# Autodesk Inventor assembly: 1Ufullsystem
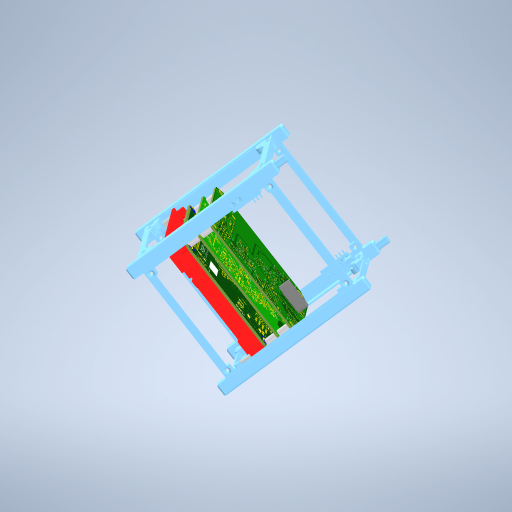
[picture p0: Inventor's stored thumbnail of the model, 512x512]
Saved by Autodesk Inventor 2024 (Build 280153000, 153)
## iProperties
Created: 2023-04-12
Part Number: 1Ufullsystem
Document SubType Name: Assembly
Designer: User
Author: User
## Documents named in this file (8)
- C:\Users\User\Documents\1UFrame\1Ufullsystem.iam
- C:\Users\User\Documents\1UFrame\ISISpace\ISIS CubeSat STS PC104 Skeleton.iam
- C:\Users\User\Documents\1UFrame\CAD_backup_frequent_files_20200629 (1)\PCB_LT_ICR.iam
- C:\Users\User\Documents\1UFrame\CAD_backup_frequent_files_20200629 (1)\PCB_LT_RX-TX.iam
- C:\Users\User\Documents\1UFrame\CAD_backup_frequent_files_20200629 (1)\PCB_LIHU.iam
- C:\Users\User\Documents\1UFrame\CAD_backup_frequent_files_20200629 (1)\standoff815mm.ipt
- C:\Users\User\Documents\1UFrame\Standoff0.335in.ipt
- C:\Users\User\Documents\1UFrame\PC104_EM-113 Assembly.iam
## Components (17 placed, 7 different names)
1. ISIS CubeSat STS PC104 Skeleton:1 [sub-assembly] — Mate:1, Mate:2, Mate:3, Mate:4
2. PCB_LT_ICR:1 [sub-assembly] — Mate:16, Mate:17, Mate:18, Mate:19, Mate:20, Mate:21, Mate:22, Mate:23
3. PCB_LT_RX-TX:1 [sub-assembly] — Mate:24, Mate:25, Mate:26, Mate:27, Mate:28, Mate:29, Mate:31, Mate:32, Mate:33, Mate:34, Mate:36, Mate:39, Mate:40
4. PCB_LIHU:2 [sub-assembly] — Mate:41, Mate:42, Mate:43, Mate:44, Mate:45, Mate:46, Mate:47, Mate:48, Mate:49, Mate:50
5. standoff815mm:1 — Mate:18, Mate:19, Mate:25, Mate:30, Mate:38
6. standoff815mm:2 — Mate:31, Mate:32, Mate:37, Mate:41, Mate:45
7. standoff815mm:3 — Mate:33, Mate:34, Mate:35, Mate:43
8. standoff815mm:4 — Mate:29, Mate:30, Mate:38, Mate:44
9. standoff815mm:5 — Mate:22, Mate:23, Mate:24, Mate:28, Mate:36
10. standoff815mm:6 — Mate:16, Mate:17, Mate:26, Mate:37
11. standoff815mm:7 — Mate:20, Mate:21, Mate:27, Mate:35
12. Standoff0.335in:1 — Mate:4, Mate:53, Mate:56, Mate:57
13. Standoff0.335in:2 — Mate:1, Mate:54, Mate:55
14. Standoff0.335in:3 — Mate:3, Mate:51, Mate:52, Mate:58
15. Standoff0.335in:4 — Mate:2, Mate:59, Mate:60
16. standoff815mm:13 — Mate:39, Mate:40, Mate:42
17. PC104_EM-113 Assembly:1 [sub-assembly] — Mate:46, Mate:47, Mate:48, Mate:49, Mate:50, Mate:51, Mate:52, Mate:53, Mate:54, Mate:55, Mate:56, Mate:57, Mate:58, Mate:59, Mate:60
## Relationships (49: Mate 49)
- Mate:1: ISIS CubeSat STS PC104 Skeleton:1 ↔ Standoff0.335in:2
- Mate:2: ISIS CubeSat STS PC104 Skeleton:1 ↔ Standoff0.335in:4
- Mate:3: ISIS CubeSat STS PC104 Skeleton:1 ↔ Standoff0.335in:3
- Mate:4: ISIS CubeSat STS PC104 Skeleton:1 ↔ Standoff0.335in:1
- Mate:16: PCB_LT_ICR:1 ↔ standoff815mm:6
- Mate:17: PCB_LT_ICR:1 ↔ standoff815mm:6
- Mate:18: PCB_LT_ICR:1 ↔ standoff815mm:1
- Mate:19: PCB_LT_ICR:1 ↔ standoff815mm:1
- Mate:20: PCB_LT_ICR:1 ↔ standoff815mm:7
- Mate:21: PCB_LT_ICR:1 ↔ standoff815mm:7
- Mate:22: PCB_LT_ICR:1 ↔ standoff815mm:5
- Mate:23: PCB_LT_ICR:1 ↔ standoff815mm:5
- Mate:24: PCB_LT_RX-TX:1 ↔ standoff815mm:5
- Mate:25: PCB_LT_RX-TX:1 ↔ standoff815mm:1
- Mate:26: PCB_LT_RX-TX:1 ↔ standoff815mm:6
- Mate:27: PCB_LT_RX-TX:1 ↔ standoff815mm:7
- Mate:28: PCB_LT_RX-TX:1 ↔ standoff815mm:5
- Mate:29: PCB_LT_RX-TX:1 ↔ standoff815mm:4
- Mate:30: standoff815mm:1 ↔ standoff815mm:4
- Mate:31: PCB_LT_RX-TX:1 ↔ standoff815mm:2
- Mate:32: PCB_LT_RX-TX:1 ↔ standoff815mm:2
- Mate:33: PCB_LT_RX-TX:1 ↔ standoff815mm:3
- Mate:34: PCB_LT_RX-TX:1 ↔ standoff815mm:3
- Mate:35: standoff815mm:3 ↔ standoff815mm:7
- Mate:36: PCB_LT_RX-TX:1 ↔ standoff815mm:5
- Mate:37: standoff815mm:2 ↔ standoff815mm:6
- Mate:38: standoff815mm:1 ↔ standoff815mm:4
- Mate:39: PCB_LT_RX-TX:1 ↔ standoff815mm:13
- Mate:40: PCB_LT_RX-TX:1 ↔ standoff815mm:13
- Mate:41: PCB_LIHU:2 ↔ standoff815mm:2
- Mate:42: PCB_LIHU:2 ↔ standoff815mm:13
- Mate:43: PCB_LIHU:2 ↔ standoff815mm:3
- Mate:44: PCB_LIHU:2 ↔ standoff815mm:4
- Mate:45: PCB_LIHU:2 ↔ standoff815mm:2
- Mate:46: PCB_LIHU:2 ↔ PC104_EM-113 Assembly:1
- Mate:47: PCB_LIHU:2 ↔ PC104_EM-113 Assembly:1
- Mate:48: PCB_LIHU:2 ↔ PC104_EM-113 Assembly:1
- Mate:49: PCB_LIHU:2 ↔ PC104_EM-113 Assembly:1
- Mate:50: PCB_LIHU:2 ↔ PC104_EM-113 Assembly:1
- Mate:51: Standoff0.335in:3 ↔ PC104_EM-113 Assembly:1
- Mate:52: Standoff0.335in:3 ↔ PC104_EM-113 Assembly:1
- Mate:53: Standoff0.335in:1 ↔ PC104_EM-113 Assembly:1
- Mate:54: Standoff0.335in:2 ↔ PC104_EM-113 Assembly:1
- Mate:55: Standoff0.335in:2 ↔ PC104_EM-113 Assembly:1
- Mate:56: Standoff0.335in:1 ↔ PC104_EM-113 Assembly:1
- Mate:57: Standoff0.335in:1 ↔ PC104_EM-113 Assembly:1
- Mate:58: Standoff0.335in:3 ↔ PC104_EM-113 Assembly:1
- Mate:59: Standoff0.335in:4 ↔ PC104_EM-113 Assembly:1
- Mate:60: Standoff0.335in:4 ↔ PC104_EM-113 Assembly:1
